# Autodesk Inventor assembly: Trunk_servo_bottom_frame_WearingImage
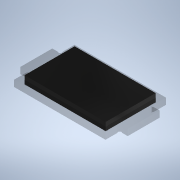
[picture p0: Inventor's stored thumbnail of the model, 180x180]
Saved by Autodesk Inventor 2022 (Build 260153000, 153)
## iProperties
Created: 2022-03-17
Part Number: Trunk_servo_bottom_frame_WearingImage
Document SubType Name: Assembly
Designer: MasatoKubotera
Author: MasatoKubotera
## Documents named in this file (3)
- C:\Users\Masato\Documents\Inventor\CIT Brains_Inventor\SUSTAINA-OP\OptionParts\SandBlastingJig\Trunk_servo_bottom_frame_WearingImage.iam
- C:\Users\Masato\Documents\Inventor\CIT Brains_Inventor\SUSTAINA-OP\UpperBody\Trunk\Trunk_servo_bottom_frame.ipt
- C:\Users\Masato\Documents\Inventor\CIT Brains_Inventor\SUSTAINA-OP\OptionParts\SandBlastingJig\Trunk_servo_bottom_frame_SandBlastingJig.ipt
## Components (2 placed, 2 different names)
1. Trunk_servo_bottom_frame:1 — メイト:1, メイト:2, メイト:3
2. Trunk_servo_bottom_frame_SandBlastingJig:1 — メイト:1, メイト:2, メイト:3
## Relationships (3: Mate 3)
- メイト:1 [Mate]: Trunk_servo_bottom_frame:1 ↔ Trunk_servo_bottom_frame_SandBlastingJig:1
- メイト:2 [Mate] (0.075 mm): Trunk_servo_bottom_frame:1 ↔ Trunk_servo_bottom_frame_SandBlastingJig:1
- メイト:3 [Mate] (0.075 mm): Trunk_servo_bottom_frame:1 ↔ Trunk_servo_bottom_frame_SandBlastingJig:1
